# Autodesk Inventor assembly: Durometer_Electronics_Enclosure_Assembly
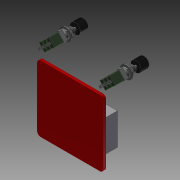
[picture p0: Inventor's stored thumbnail of the model, 180x180]
Saved by Autodesk Inventor 2015 (Build 190159000, 159)
## iProperties
Created: 2015-01-04
Part Number: Durometer_Electronics_Enclosure_Assembly
Document SubType Name: Assembly
Designer: Drew
Author: Drew
## Documents named in this file (5)
- C:\Users\Drew\Dropbox\Durometer\Durometer_Assembly\Durometer_Electronics_Enclosure_Assembly.iam
- C:\Users\Drew\Dropbox\Durometer\Durometer_Assembly\Durometer_Electronics_Enclosure.ipt
- C:\Users\Drew\Dropbox\Durometer\Durometer_Assembly\Arduino_pro_mini.iam
- C:\Users\Drew\Dropbox\Durometer\Durometer_Assembly\Big_Easy_Stepper_Driver.ipt
- C:\Users\Drew\Dropbox\Durometer\Durometer_Assembly\MB2011SS1W01_CA.iam
## Components (5 placed, 4 different names)
1. Durometer_Electronics_Enclosure:1 — Mate:1, Mate:2, Flush:1, Flush:2
2. Arduino_pro_mini:1 [sub-assembly] — Mate:2, Flush:1
3. Big_Easy_Stepper_Driver:1 — Mate:1, Flush:2
4. MB2011SS1W01_CA:1 [sub-assembly]
5. MB2011SS1W01_CA:2 [sub-assembly]
## Relationships (4: Mate 2, Flush 2)
- Mate:1: Durometer_Electronics_Enclosure:1 ↔ Big_Easy_Stepper_Driver:1
- Mate:2: Durometer_Electronics_Enclosure:1 ↔ Arduino_pro_mini:1
- Flush:1 (3.81 mm): Durometer_Electronics_Enclosure:1 ↔ Arduino_pro_mini:1
- Flush:2 (3.81 mm): Durometer_Electronics_Enclosure:1 ↔ Big_Easy_Stepper_Driver:1
